# Autodesk Inventor assembly: Pickup
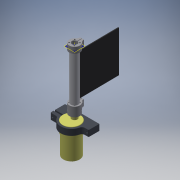
[picture p0: Inventor's stored thumbnail of the model, 180x180]
Saved by Autodesk Inventor 2016 (Build 200138000, 138)
## iProperties
Created: 2015-11-25
Part Number: Pickup
Document SubType Name: Assembly
Designer: Julia
Author: Julia
## Documents named in this file (6)
- C:\Users\Julia\Documents\GitHub\RobotuxCAD\FTC CAD Parts\Pickup.iam
- C:\Users\Julia\Documents\GitHub\RobotuxCAD\FTC CAD Parts\Pickup Motor.iam
- C:\Users\Julia\Documents\GitHub\RobotuxCAD\FTC CAD Parts\Pickup Pvc.ipt
- C:\Users\Julia\Documents\GitHub\RobotuxCAD\FTC CAD Parts\Pickup Rubber.ipt
- C:\Users\Julia\Documents\GitHub\RobotuxCAD\FTC CAD Parts\tube_clamp_2012.ipt
- C:\Users\Julia\Documents\GitHub\RobotuxCAD\FTC CAD Parts\Tetrix_Kit_FTC\tetrix_739079_collar_2012.ipt
## Components (6 placed, 5 different names)
1. Pickup Motor:1 [sub-assembly] — Mate:1, Mate:2, Mate:4, Mate:6, Mate:12
2. Pickup Pvc:1 — Mate:5, Mate:6, Mate:7, Mate:8, Mate:9, Mate:10, Mate:11, Mate:12, Mate:13, Mate:14
3. Pickup Rubber:1 — Mate:13, Mate:14
4. tube_clamp_2012:1 — Mate:3, Mate:4, Mate:5, Mate:11
5. tube_clamp_2012:2 — Mate:7, Mate:8, Mate:9, Mate:10
6. tetrix_739079_collar_2012:1 — Mate:1, Mate:2, Mate:3
## Relationships (14: Mate 14)
- Mate:1: Pickup Motor:1 ↔ tetrix_739079_collar_2012:1
- Mate:2: Pickup Motor:1 ↔ tetrix_739079_collar_2012:1
- Mate:3: tube_clamp_2012:1 ↔ tetrix_739079_collar_2012:1
- Mate:4: Pickup Motor:1 ↔ tube_clamp_2012:1
- Mate:5: Pickup Pvc:1 ↔ tube_clamp_2012:1
- Mate:6: Pickup Motor:1 ↔ Pickup Pvc:1
- Mate:7: Pickup Pvc:1 ↔ tube_clamp_2012:2
- Mate:8: Pickup Pvc:1 ↔ tube_clamp_2012:2
- Mate:9: Pickup Pvc:1 ↔ tube_clamp_2012:2
- Mate:10: Pickup Pvc:1 ↔ tube_clamp_2012:2
- Mate:11: Pickup Pvc:1 ↔ tube_clamp_2012:1
- Mate:12: Pickup Motor:1 ↔ Pickup Pvc:1
- Mate:13: Pickup Pvc:1 ↔ Pickup Rubber:1
- Mate:14: Pickup Pvc:1 ↔ Pickup Rubber:1
